# Autodesk Inventor assembly: XY Idle Belt Holder
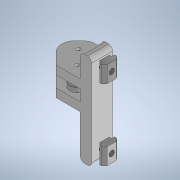
[picture p0: Inventor's stored thumbnail of the model, 180x180]
Saved by Autodesk Inventor 2022 (Build 260153000, 153)
## iProperties
Created: 2022-03-12
Part Number: XY Idle Belt Holder
Document SubType Name: Assembly
Designer: Nick
Author: Nick
## Documents named in this file (6)
- Y:\Projects\Bibble0\SubAsm\XY Idle Belt Holder.iam
- Y:\Projects\Bibble0\Hardware\M3 T-Slot Nut.ipt
- Y:\Projects\Bibble0\Bearings\603 Bearing.ipt
- Y:\Projects\Bibble0\3D printed\X-Y Axis\Idle Belt Holder.ipt
- Y:\Projects\Bibble0\Hardware\M3 x 8 mm SHCS.ipt
- Y:\Projects\Bibble0\Hardware\M3 x 16 mm SS.ipt
## Components (11 placed, 5 different names)
1. M3 T-Slot Nut:1 — Insert:4, Angle:2
2. M3 T-Slot Nut:2 — Insert:3, Angle:1, Angle:2
3. 603 Bearing:1 — Insert:5
4. 603 Bearing:2 — Insert:5, Insert:8
5. 603 Bearing:3 — Insert:6
6. 603 Bearing:4 — Insert:6, Insert:7
7. Idle Belt Holder:1 — Insert:1, Insert:2, Insert:3, Insert:4, Angle:1, Insert:7, Insert:8, Insert:9, Insert:10
8. M3 x 8 mm SHCS:1 — Insert:1
9. M3 x 8 mm SHCS:2 — Insert:2
10. M3 x 16 mm SS:1 — Insert:9
11. M3 x 16 mm SS:2 — Insert:10
## Relationships (12: Insert 10, Angle 2)
- Insert:1: Idle Belt Holder:1 ↔ M3 x 8 mm SHCS:1
- Insert:2: Idle Belt Holder:1 ↔ M3 x 8 mm SHCS:2
- Insert:3 (1.5 mm): M3 T-Slot Nut:2 ↔ Idle Belt Holder:1
- Insert:4 (1.5 mm): M3 T-Slot Nut:1 ↔ Idle Belt Holder:1
- Angle:1 (0 deg): M3 T-Slot Nut:2 ↔ Idle Belt Holder:1
- Angle:2 (0 deg): M3 T-Slot Nut:1 ↔ M3 T-Slot Nut:2
- Insert:5: 603 Bearing:1 ↔ 603 Bearing:2
- Insert:6: 603 Bearing:3 ↔ 603 Bearing:4
- Insert:7 (0.5 mm): 603 Bearing:4 ↔ Idle Belt Holder:1
- Insert:8 (0.5 mm): 603 Bearing:2 ↔ Idle Belt Holder:1
- Insert:9: Idle Belt Holder:1 ↔ M3 x 16 mm SS:1
- Insert:10: Idle Belt Holder:1 ↔ M3 x 16 mm SS:2
